# Autodesk Inventor assembly: gimbal_assembly_2
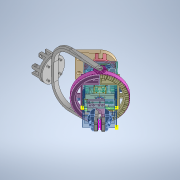
[picture p0: Inventor's stored thumbnail of the model, 180x180]
Saved by Autodesk Inventor 2022 (Build 260153000, 153)
## iProperties
Created: 2022-03-15
Part Number: gimbal_assembly_2
Document SubType Name: Assembly
Designer: kylem
Author: kylem
## Documents named in this file (8)
- C:\Users\kylem\OneDrive\Documents\GitHub\IMML_Contactile_Gripper_Hardware\gimbal_assembly_2.iam
- C:\Users\kylem\OneDrive\Documents\GitHub\IMML_Contactile_Gripper_Hardware\Gripper_Design_NonCompliant_No_UR5.iam
- C:\Users\kylem\OneDrive\Documents\GitHub\IMML_Contactile_Gripper_Hardware\test_stand\gripper_mount_female.ipt
- C:\Users\kylem\OneDrive\Documents\GitHub\IMML_Contactile_Gripper_Hardware\test_stand\gripper_mount_male.ipt
- C:\Users\kylem\OneDrive\Documents\GitHub\IMML_Contactile_Gripper_Hardware\test_stand\gripper_mount_ring.ipt
- C:\Users\kylem\OneDrive\Documents\GitHub\IMML_Contactile_Gripper_Hardware\test_stand\gimbal_ring_second.ipt
- C:\Users\kylem\OneDrive\Documents\GitHub\IMML_Contactile_Gripper_Hardware\gimbal_base_mount_2.ipt
- C:\Users\kylem\OneDrive\Documents\GitHub\IMML_Contactile_Gripper_Hardware\bottom_gimbal_ring_2.ipt
## Components (7 placed, 7 different names)
1. Gripper_Design_NonCompliant_No_UR5:1 [sub-assembly] — Mate:12, Mate:13, Mate:14, Mate:17, Angle:3
2. gripper_mount_female:1 — Mate:12, Mate:13, Mate:14, Mate:15, Mate:16, Mate:23
3. gripper_mount_male:1 — Mate:15, Mate:16, Mate:17, Mate:22, Mate:24, Mate:26
4. gripper_mount_ring:1 — Mate:22, Mate:24, Mate:25
5. gimbal_ring_second:1 — Mate:23, Mate:25, Mate:26, Mate:27, Mate:28
6. gimbal_base_mount_2:1 — Mate:29, Mate:30, Mate:31, Mate:32, Mate:33, Mate:34, Angle:1
7. bottom_gimbal_ring_2:1 — Mate:27, Mate:28, Mate:29, Mate:30, Mate:31, Angle:3
## Relationships (21: Mate 19, Angle 2)
- Mate:12: Gripper_Design_NonCompliant_No_UR5:1 ↔ gripper_mount_female:1
- Mate:13: Gripper_Design_NonCompliant_No_UR5:1 ↔ gripper_mount_female:1
- Mate:14: Gripper_Design_NonCompliant_No_UR5:1 ↔ gripper_mount_female:1
- Mate:15: gripper_mount_female:1 ↔ gripper_mount_male:1
- Mate:16: gripper_mount_female:1 ↔ gripper_mount_male:1
- Mate:17: Gripper_Design_NonCompliant_No_UR5:1 ↔ gripper_mount_male:1
- Mate:22: gripper_mount_male:1 ↔ gripper_mount_ring:1
- Mate:23: gripper_mount_female:1 ↔ gimbal_ring_second:1
- Mate:24: gripper_mount_male:1 ↔ gripper_mount_ring:1
- Mate:25: gripper_mount_ring:1 ↔ gimbal_ring_second:1
- Mate:26 (0.25 mm): gripper_mount_male:1 ↔ gimbal_ring_second:1
- Mate:27: gimbal_ring_second:1 ↔ bottom_gimbal_ring_2:1
- Mate:28: gimbal_ring_second:1 ↔ bottom_gimbal_ring_2:1
- Mate:29: gimbal_base_mount_2:1 ↔ bottom_gimbal_ring_2:1
- Mate:30: gimbal_base_mount_2:1 ↔ bottom_gimbal_ring_2:1
- Mate:31: gimbal_base_mount_2:1 ↔ bottom_gimbal_ring_2:1
- Mate:32: gimbal_base_mount_2:1
- Mate:33: gimbal_base_mount_2:1
- Mate:34: gimbal_base_mount_2:1
- Angle:1 (0 deg): gimbal_base_mount_2:1
- Angle:3 (0 deg): Gripper_Design_NonCompliant_No_UR5:1 ↔ bottom_gimbal_ring_2:1
